# Autodesk Inventor assembly: tesaki_arata
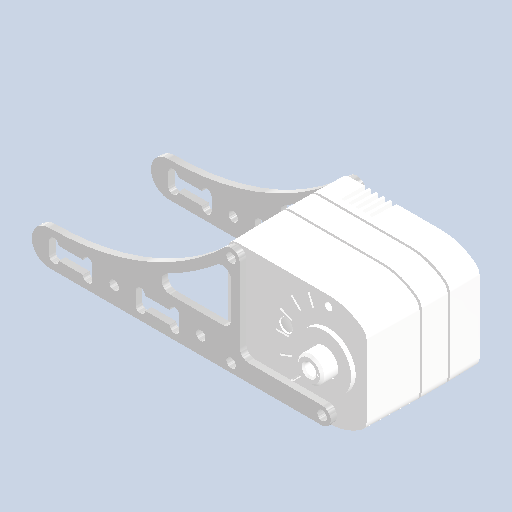
[picture p0: Inventor's stored thumbnail of the model, 512x512]
Saved by Autodesk Inventor 2024 (Build 280153000, 153)
## iProperties
Created: 2024-01-03
Part Number: tesaki_arata
Document SubType Name: Assembly
Designer: right
Mass: 38.2211 g
Surface Area: 100.453 cm^2
Volume: 22.6663 cm^3
Density: 1.68625 g/cm^3
Author: right
## Documents named in this file (3)
- C:\Users\right\OneDrive\ドキュメント\Inventor\V2二足Light＿仮\tesaki_arata.iam
- C:\Users\right\OneDrive\ドキュメント\Inventor\V2二足Light＿仮\KRS3300_scale.ipt
- C:\Users\right\OneDrive\ドキュメント\Inventor\V2二足Light＿仮\3304_tesaki.ipt
## Components (3 placed, 2 different names)
1. KRS3300_scale:1 — フラッシュ:1, 挿入:3, 挿入:4, 挿入:5, 挿入:6
2. 3304_tesaki:1 — フラッシュ:1, 挿入:3, 挿入:4
3. 3304_tesaki:2 — 挿入:5, 挿入:6
## Relationships (5: Insert 4, Flush 1)
- フラッシュ:1 [Flush]: KRS3300_scale:1 ↔ 3304_tesaki:1
- 挿入:3 [Insert]: KRS3300_scale:1 ↔ 3304_tesaki:1
- 挿入:4 [Insert]: KRS3300_scale:1 ↔ 3304_tesaki:1
- 挿入:5 [Insert]: KRS3300_scale:1 ↔ 3304_tesaki:2
- 挿入:6 [Insert]: KRS3300_scale:1 ↔ 3304_tesaki:2
